# Autodesk Inventor assembly: Balloon Assembly
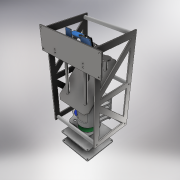
[picture p0: Inventor's stored thumbnail of the model, 180x180]
Saved by Autodesk Inventor 2017 (Build 210142000, 142)
## iProperties
Created: 2017-04-01
Part Number: Balloon Assembly
Document SubType Name: Assembly
Designer: Muchen
Author: Muchen
## Documents named in this file (14)
- F:\OneDrive\Documents\2017 UBC\UBC Orbit\Payload\Balloon Test\Balloon Assembly.iam
- F:\OneDrive\Documents\2017 UBC\UBC Orbit\Payload\Balloon Test\STEPPER MOTOR MOUNT.ipt
- F:\OneDrive\Documents\2017 UBC\UBC Orbit\Payload\Balloon Test\STEPPER MOTOR.ipt
- F:\OneDrive\Documents\2017 UBC\UBC Orbit\Payload\Balloon Test\MIRROR MOUNT.ipt
- F:\OneDrive\Documents\2017 UBC\UBC Orbit\Payload\Balloon Test\BASE.ipt
- F:\OneDrive\Documents\2017 UBC\UBC Orbit\Payload\Balloon Test\INFORCE.ipt
- F:\OneDrive\Documents\2017 UBC\UBC Orbit\Payload\Balloon Test\CAMERA.ipt
- F:\OneDrive\Documents\2017 UBC\UBC Orbit\Payload\Balloon Test\LENS.ipt
- F:\OneDrive\Documents\2017 UBC\UBC Orbit\Payload\Balloon Test\LENS MOUNT.ipt
- F:\OneDrive\Documents\2017 UBC\UBC Orbit\Payload\Balloon Test\MICROCONTROLLER.ipt
- F:\OneDrive\Documents\2017 UBC\UBC Orbit\Payload\Balloon Test\STEPPER DRIVER.ipt
- F:\OneDrive\Documents\2017 UBC\UBC Orbit\Payload\Balloon Test\IMU SENSOR.ipt
- F:\OneDrive\Documents\2017 UBC\UBC Orbit\Payload\Balloon Test\FILTER WHEEL.ipt
- F:\OneDrive\Documents\2017 UBC\UBC Orbit\Payload\Balloon Test\LONG STANDOFFS.ipt
## Components (16 placed, 13 different names)
1. STEPPER MOTOR MOUNT:1 — Mate:2, Angle:1, Mate:3, Mate:8, Mate:9, Mate:10
2. STEPPER MOTOR:1 — Mate:2, Angle:1, Mate:3, Mate:4, Mate:11, Mate:19
3. MIRROR MOUNT:1 — Mate:4, Mate:11
4. BASE:1 — Mate:8, Mate:9, Mate:10, Mate:21, Mate:22, Mate:23, Mate:24, Mate:25, Mate:26, Mate:27, Mate:28
5. INFORCE:1 — Mate:12, Mate:13
6. CAMERA:1 — Mate:12, Mate:13, Mate:14, Mate:15
7. LENS:1 — Mate:14, Mate:15, Mate:16, Mate:20
8. LENS MOUNT:1 — Mate:16, Mate:19
9. MICROCONTROLLER:1
10. STEPPER DRIVER:1
11. IMU SENSOR:1
12. FILTER WHEEL:1 — Mate:20
13. LONG STANDOFFS:1 — Mate:21, Mate:25
14. LONG STANDOFFS:2 — Mate:22, Mate:26
15. LONG STANDOFFS:3 — Mate:23, Mate:27
16. LONG STANDOFFS:4 — Mate:24, Mate:28
## Relationships (23: Mate 22, Angle 1)
- Mate:2: STEPPER MOTOR MOUNT:1 ↔ STEPPER MOTOR:1
- Angle:1 (0 deg): STEPPER MOTOR MOUNT:1 ↔ STEPPER MOTOR:1
- Mate:3: STEPPER MOTOR MOUNT:1 ↔ STEPPER MOTOR:1
- Mate:4: STEPPER MOTOR:1 ↔ MIRROR MOUNT:1
- Mate:8: STEPPER MOTOR MOUNT:1 ↔ BASE:1
- Mate:9: STEPPER MOTOR MOUNT:1 ↔ BASE:1
- Mate:10: STEPPER MOTOR MOUNT:1 ↔ BASE:1
- Mate:11: STEPPER MOTOR:1 ↔ MIRROR MOUNT:1
- Mate:12: INFORCE:1 ↔ CAMERA:1
- Mate:13: INFORCE:1 ↔ CAMERA:1
- Mate:14: CAMERA:1 ↔ LENS:1
- Mate:15 (35 mm): CAMERA:1 ↔ LENS:1
- Mate:16: LENS:1 ↔ LENS MOUNT:1
- Mate:19: STEPPER MOTOR:1 ↔ LENS MOUNT:1
- Mate:20: LENS:1 ↔ FILTER WHEEL:1
- Mate:21: BASE:1 ↔ LONG STANDOFFS:1
- Mate:22: BASE:1 ↔ LONG STANDOFFS:2
- Mate:23: BASE:1 ↔ LONG STANDOFFS:3
- Mate:24: BASE:1 ↔ LONG STANDOFFS:4
- Mate:25: BASE:1 ↔ LONG STANDOFFS:1
- Mate:26: BASE:1 ↔ LONG STANDOFFS:2
- Mate:27: BASE:1 ↔ LONG STANDOFFS:3
- Mate:28: BASE:1 ↔ LONG STANDOFFS:4
